# Autodesk Inventor assembly: Projectile Launcher Design 1
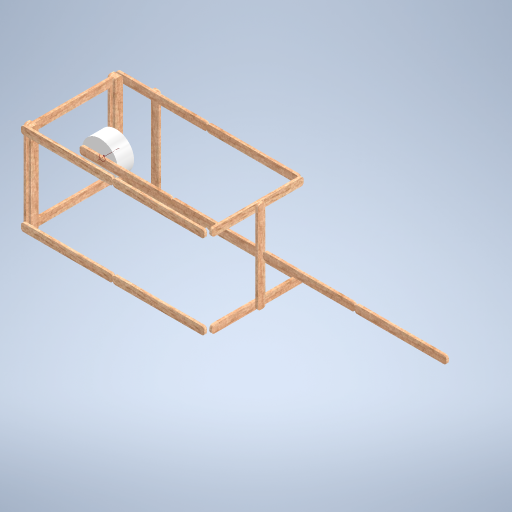
[picture p0: Inventor's stored thumbnail of the model, 512x512]
Saved by Autodesk Inventor 2024 (Build 280153000, 153)
## iProperties
Created: 2023-09-15
Part Number: Projectile Launcher Design 1
Document SubType Name: Assembly
Designer: Nick
Author: Nick
## Documents named in this file (5)
- C:\Users\Nick\Documents\Inventor\MMAE 100\Projectile Launcher Design 1.iam
- C:\Users\Nick\Documents\Inventor\MMAE 100\Projectile Launcher Popsicle Stick.ipt
- C:\Users\Nick\Documents\Inventor\MMAE 100\Projectile Launcher Popsicle Stick_MIR.ipt
- C:\Users\Nick\Documents\Inventor\MMAE 100\Projectile Launcher Popsicle Stick_MIR1.ipt
- C:\Users\Nick\Documents\Inventor\MMAE 100\Projectile Launcher Ball Holder.ipt
## Components (24 placed, 4 different names)
1. Projectile Launcher Popsicle Stick:1 — Mate:1, Flush:1, Flush:2, Flush:5, Flush:6, Flush:36, Mate:24, Mate:25
2. Projectile Launcher Popsicle Stick:2 — Mate:5, Flush:9, Flush:10, Mate:6, Mate:7
3. Projectile Launcher Popsicle Stick:3 — Flush:5, Mate:3, Flush:6, Mate:4, Flush:7, Flush:8, Flush:9, Flush:10, Flush:11
4. Projectile Launcher Popsicle Stick:4 — Mate:1, Flush:1, Flush:2, Mate:2, Flush:3, Flush:4, Mate:5, Flush:13, Flush:45
5. Projectile Launcher Popsicle Stick:5 — Mate:4, Flush:7, Flush:8, Flush:12, Flush:14
6. Projectile Launcher Popsicle Stick:6 — Mate:2, Flush:3, Flush:4, Mate:3, Flush:46, Flush:47
7. Projectile Launcher Popsicle Stick:7 — Mate:15, Flush:28, Flush:29
8. Projectile Launcher Popsicle Stick:8 — Mate:13, Flush:24, Flush:25, Mate:14, Flush:26, Flush:27, Flush:32
9. Projectile Launcher Popsicle Stick:9 — Mate:13, Flush:24, Flush:25, Mate:22, Tangent:1, Tangent:2
10. Projectile Launcher Popsicle Stick:13 — Mate:14, Flush:26, Flush:27, Mate:15, Flush:28, Flush:29, Mate:17, Flush:33
11. Projectile Launcher Popsicle Stick:14 — Flush:20, Flush:21, Mate:10, Mate:12, Flush:22, Flush:23
12. Projectile Launcher Popsicle Stick:15 — Mate:18, Flush:34, Flush:35
13. Projectile Launcher Popsicle Stick:16 — Mate:12, Flush:22, Flush:23
14. Projectile Launcher Popsicle Stick:17 — Flush:15, Mate:8, Flush:16, Flush:20, Flush:21, Mate:10
15. Projectile Launcher Popsicle Stick:18 — Mate:6, Flush:11, Flush:12, Flush:17, Mate:9, Flush:18, Flush:19, Mate:11, Mate:18, Flush:34, Flush:35
16. Projectile Launcher Popsicle Stick:19 — Mate:7, Flush:13, Flush:14, Flush:15, Mate:8, Flush:16
17. Projectile Launcher Popsicle Stick:20 — Flush:17, Mate:9, Flush:18, Flush:19, Flush:37, Mate:23, Flush:43, Flush:44
18. Projectile Launcher Popsicle Stick_MIR:1 — Flush:30, Flush:31, Mate:16, Flush:33, Flush:37, Mate:23, Flush:43, Flush:44
19. Projectile Launcher Popsicle Stick_MIR:2 — Flush:30, Flush:31, Mate:16, Mate:17, Flush:32
20. Projectile Launcher Popsicle Stick_MIR1:1 — Flush:38, Mate:20, Flush:39, Mate:24, Flush:45
21. Projectile Launcher Popsicle Stick_MIR1:2 — Mate:19, Flush:40, Flush:41, Mate:21, Flush:42, Mate:25, Flush:47
22. Projectile Launcher Popsicle Stick_MIR1:3 — Flush:38, Mate:20, Flush:39, Flush:46
23. Projectile Launcher Popsicle Stick_MIR1:4 — Flush:40, Flush:41, Mate:21, Flush:42
24. Projectile Launcher Ball Holder:1 — Mate:22, Tangent:1, Tangent:2
## Relationships (74: Flush 47, Mate 25, Tangent 2)
- Mate:1: Projectile Launcher Popsicle Stick:1 ↔ Projectile Launcher Popsicle Stick:4
- Flush:1: Projectile Launcher Popsicle Stick:1 ↔ Projectile Launcher Popsicle Stick:4
- Flush:2: Projectile Launcher Popsicle Stick:1 ↔ Projectile Launcher Popsicle Stick:4
- Mate:2: Projectile Launcher Popsicle Stick:4 ↔ Projectile Launcher Popsicle Stick:6
- Flush:3: Projectile Launcher Popsicle Stick:4 ↔ Projectile Launcher Popsicle Stick:6
- Flush:4: Projectile Launcher Popsicle Stick:4 ↔ Projectile Launcher Popsicle Stick:6
- Flush:5: Projectile Launcher Popsicle Stick:1 ↔ Projectile Launcher Popsicle Stick:3
- Mate:3: Projectile Launcher Popsicle Stick:3 ↔ Projectile Launcher Popsicle Stick:6
- Flush:6: Projectile Launcher Popsicle Stick:1 ↔ Projectile Launcher Popsicle Stick:3
- Mate:4: Projectile Launcher Popsicle Stick:3 ↔ Projectile Launcher Popsicle Stick:5
- Flush:7: Projectile Launcher Popsicle Stick:3 ↔ Projectile Launcher Popsicle Stick:5
- Flush:8: Projectile Launcher Popsicle Stick:3 ↔ Projectile Launcher Popsicle Stick:5
- Mate:5: Projectile Launcher Popsicle Stick:2 ↔ Projectile Launcher Popsicle Stick:4
- Flush:9: Projectile Launcher Popsicle Stick:2 ↔ Projectile Launcher Popsicle Stick:3
- Flush:10: Projectile Launcher Popsicle Stick:2 ↔ Projectile Launcher Popsicle Stick:3
- Mate:6: Projectile Launcher Popsicle Stick:2 ↔ Projectile Launcher Popsicle Stick:18
- Flush:11: Projectile Launcher Popsicle Stick:3 ↔ Projectile Launcher Popsicle Stick:18
- Flush:12: Projectile Launcher Popsicle Stick:5 ↔ Projectile Launcher Popsicle Stick:18
- Mate:7: Projectile Launcher Popsicle Stick:2 ↔ Projectile Launcher Popsicle Stick:19
- Flush:13: Projectile Launcher Popsicle Stick:4 ↔ Projectile Launcher Popsicle Stick:19
- Flush:14: Projectile Launcher Popsicle Stick:5 ↔ Projectile Launcher Popsicle Stick:19
- Flush:15: Projectile Launcher Popsicle Stick:17 ↔ Projectile Launcher Popsicle Stick:19
- Mate:8: Projectile Launcher Popsicle Stick:17 ↔ Projectile Launcher Popsicle Stick:19
- Flush:16: Projectile Launcher Popsicle Stick:17 ↔ Projectile Launcher Popsicle Stick:19
- Flush:17: Projectile Launcher Popsicle Stick:18 ↔ Projectile Launcher Popsicle Stick:20
- Mate:9: Projectile Launcher Popsicle Stick:18 ↔ Projectile Launcher Popsicle Stick:20
- Flush:18: Projectile Launcher Popsicle Stick:18 ↔ Projectile Launcher Popsicle Stick:20
- Flush:19: Projectile Launcher Popsicle Stick:18 ↔ Projectile Launcher Popsicle Stick:20
- Flush:20: Projectile Launcher Popsicle Stick:14 ↔ Projectile Launcher Popsicle Stick:17
- Flush:21: Projectile Launcher Popsicle Stick:14 ↔ Projectile Launcher Popsicle Stick:17
- Mate:10: Projectile Launcher Popsicle Stick:14 ↔ Projectile Launcher Popsicle Stick:17
- Mate:11 (47.625 mm): Projectile Launcher Popsicle Stick:18
- Mate:12: Projectile Launcher Popsicle Stick:14 ↔ Projectile Launcher Popsicle Stick:16
- Flush:22: Projectile Launcher Popsicle Stick:14 ↔ Projectile Launcher Popsicle Stick:16
- Flush:23 (50.8 mm): Projectile Launcher Popsicle Stick:14 ↔ Projectile Launcher Popsicle Stick:16
- Mate:13: Projectile Launcher Popsicle Stick:8 ↔ Projectile Launcher Popsicle Stick:9
- Flush:24: Projectile Launcher Popsicle Stick:8 ↔ Projectile Launcher Popsicle Stick:9
- Flush:25: Projectile Launcher Popsicle Stick:8 ↔ Projectile Launcher Popsicle Stick:9
- Mate:14: Projectile Launcher Popsicle Stick:8 ↔ Projectile Launcher Popsicle Stick:13
- Flush:26: Projectile Launcher Popsicle Stick:8 ↔ Projectile Launcher Popsicle Stick:13
- Flush:27: Projectile Launcher Popsicle Stick:8 ↔ Projectile Launcher Popsicle Stick:13
- Mate:15: Projectile Launcher Popsicle Stick:7 ↔ Projectile Launcher Popsicle Stick:13
- Flush:28: Projectile Launcher Popsicle Stick:7 ↔ Projectile Launcher Popsicle Stick:13
- Flush:29: Projectile Launcher Popsicle Stick:7 ↔ Projectile Launcher Popsicle Stick:13
- Flush:30 (50.8 mm): Projectile Launcher Popsicle Stick_MIR:1 ↔ Projectile Launcher Popsicle Stick_MIR:2
- Flush:31: Projectile Launcher Popsicle Stick_MIR:1 ↔ Projectile Launcher Popsicle Stick_MIR:2
- Mate:16: Projectile Launcher Popsicle Stick_MIR:1 ↔ Projectile Launcher Popsicle Stick_MIR:2
- Mate:17: Projectile Launcher Popsicle Stick:13 ↔ Projectile Launcher Popsicle Stick_MIR:2
- Flush:32: Projectile Launcher Popsicle Stick:8 ↔ Projectile Launcher Popsicle Stick_MIR:2
- Flush:33 (52.07 mm): Projectile Launcher Popsicle Stick:13 ↔ Projectile Launcher Popsicle Stick_MIR:1
- Mate:18: Projectile Launcher Popsicle Stick:15 ↔ Projectile Launcher Popsicle Stick:18
- Flush:34: Projectile Launcher Popsicle Stick:15 ↔ Projectile Launcher Popsicle Stick:18
- Flush:35 (-63.5 mm): Projectile Launcher Popsicle Stick:15 ↔ Projectile Launcher Popsicle Stick:18
- Flush:36 (57.15 mm): Projectile Launcher Popsicle Stick:1
- Flush:37: Projectile Launcher Popsicle Stick:20 ↔ Projectile Launcher Popsicle Stick_MIR:1
- Mate:19 (47.625 mm): Projectile Launcher Popsicle Stick_MIR1:2
- Flush:38: Projectile Launcher Popsicle Stick_MIR1:1 ↔ Projectile Launcher Popsicle Stick_MIR1:3
- Mate:20: Projectile Launcher Popsicle Stick_MIR1:1 ↔ Projectile Launcher Popsicle Stick_MIR1:3
- Flush:39: Projectile Launcher Popsicle Stick_MIR1:1 ↔ Projectile Launcher Popsicle Stick_MIR1:3
- Flush:40: Projectile Launcher Popsicle Stick_MIR1:2 ↔ Projectile Launcher Popsicle Stick_MIR1:4
- Flush:41: Projectile Launcher Popsicle Stick_MIR1:2 ↔ Projectile Launcher Popsicle Stick_MIR1:4
- Mate:21: Projectile Launcher Popsicle Stick_MIR1:2 ↔ Projectile Launcher Popsicle Stick_MIR1:4
- Flush:42: Projectile Launcher Popsicle Stick_MIR1:2 ↔ Projectile Launcher Popsicle Stick_MIR1:4
- Mate:22: Projectile Launcher Popsicle Stick:9 ↔ Projectile Launcher Ball Holder:1
- Tangent:1: Projectile Launcher Popsicle Stick:9 ↔ Projectile Launcher Ball Holder:1
- Mate:23: Projectile Launcher Popsicle Stick:20 ↔ Projectile Launcher Popsicle Stick_MIR:1
- Flush:43: Projectile Launcher Popsicle Stick:20 ↔ Projectile Launcher Popsicle Stick_MIR:1
- Flush:44: Projectile Launcher Popsicle Stick:20 ↔ Projectile Launcher Popsicle Stick_MIR:1
- Mate:24: Projectile Launcher Popsicle Stick:1 ↔ Projectile Launcher Popsicle Stick_MIR1:1
- Flush:45: Projectile Launcher Popsicle Stick:4 ↔ Projectile Launcher Popsicle Stick_MIR1:1
- Flush:46: Projectile Launcher Popsicle Stick:6 ↔ Projectile Launcher Popsicle Stick_MIR1:3
- Mate:25: Projectile Launcher Popsicle Stick:1 ↔ Projectile Launcher Popsicle Stick_MIR1:2
- Flush:47: Projectile Launcher Popsicle Stick:6 ↔ Projectile Launcher Popsicle Stick_MIR1:2
- Tangent:2 (-16.51 mm): Projectile Launcher Popsicle Stick:9 ↔ Projectile Launcher Ball Holder:1
